# Autodesk Inventor assembly: Full_model
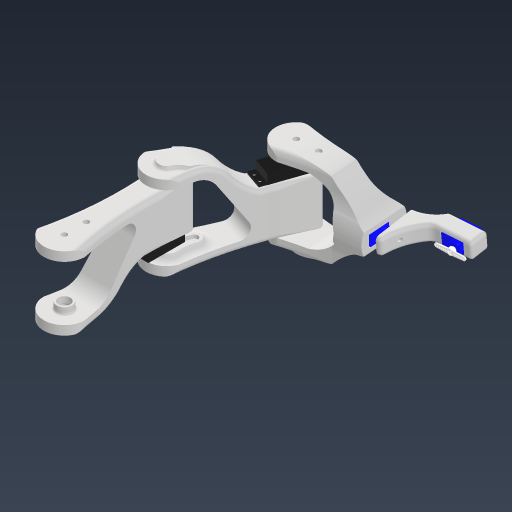
[picture p0: Inventor's stored thumbnail of the model, 512x512]
Saved by Autodesk Inventor 2024 (Build 280153000, 153)
## iProperties
Created: 2025-08-29
Part Number: Full_model
Document SubType Name: Assembly
Designer: Piter
Author: Piter
## Documents named in this file (7)
- C:\Users\Piter\OneDrive\Pulpit\Robots\david_Arm\Davie-Robot-Arm\3D Models\Full_model.iam
- C:\Users\Piter\OneDrive\Pulpit\Robots\david_Arm\Davie-Robot-Arm\3D Models\Arm1.ipt
- C:\Users\Piter\OneDrive\Pulpit\Robots\david_Arm\Davie-Robot-Arm\3D Models\Arm2.ipt
- C:\Users\Piter\OneDrive\Pulpit\Robots\david_Arm\Davie-Robot-Arm\3D Models\feetech_25kg_servo.ipt
- C:\Users\Piter\OneDrive\Pulpit\Robots\david_Arm\Davie-Robot-Arm\3D Models\Arm3.ipt
- C:\Users\Piter\OneDrive\Pulpit\Robots\david_Arm\Davie-Robot-Arm\3D Models\TowerPro SG90 M.ipt
- C:\Users\Piter\OneDrive\Pulpit\Robots\david_Arm\Davie-Robot-Arm\3D Models\Arm4.ipt
## Components (8 placed, 6 different names)
1. Arm1:1 — Rotational:1, Rotational:2
2. Arm2:1 — Rotational:2, Rigid:4, Rotational:4
3. feetech_25kg_servo:1 — Rotational:1
4. feetech_25kg_servo:2 — Rigid:4
5. Arm3:1 — Rotational:4, Rigid:1
6. TowerPro SG90 M:1 — Rigid:1, Rotational:5
7. Arm4:1 — Rotational:5, Rigid:5
8. TowerPro SG90 M:2 — Rigid:5
## Relationships (7: RevoluteJoint 4, WeldJoint 3)
- Rotational:1 [RevoluteJoint]: Arm1:1 ↔ feetech_25kg_servo:1
- Rotational:2 [RevoluteJoint]: Arm1:1 ↔ Arm2:1
- Rigid:4 [WeldJoint]: Arm2:1 ↔ feetech_25kg_servo:2
- Rotational:4 [RevoluteJoint]: Arm2:1 ↔ Arm3:1
- Rigid:1 [WeldJoint]: Arm3:1 ↔ TowerPro SG90 M:1
- Rotational:5 [RevoluteJoint]: TowerPro SG90 M:1 ↔ Arm4:1
- Rigid:5 [WeldJoint]: Arm4:1 ↔ TowerPro SG90 M:2
